# Autodesk Inventor assembly: tosaerba
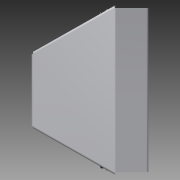
[picture p0: Inventor's stored thumbnail of the model, 180x180]
Saved by Autodesk Inventor 2014 SP2 (Build 180246200, 246)
## iProperties
Created: 2019-04-05
Part Number: tosaerba
Document SubType Name: Assembly
Designer: GauchoHP
Author: GauchoHP
## Documents named in this file (9)
- C:\Users\GauchoHP\Desktop\tosaerba\LawnmowerMechanicalProject\3D PROJECT - INVENTOR 2014\tosaerba.iam
- C:\Users\GauchoHP\Desktop\tosaerba\LawnmowerMechanicalProject\3D PROJECT - INVENTOR 2014\piastra.ipt
- C:\Users\GauchoHP\Desktop\tosaerba\LawnmowerMechanicalProject\3D PROJECT - INVENTOR 2014\motore.iam
- C:\Users\GauchoHP\Desktop\tosaerba\LawnmowerMechanicalProject\3D PROJECT - INVENTOR 2014\lama.ipt
- C:\Users\GauchoHP\Desktop\tosaerba\LawnmowerMechanicalProject\3D PROJECT - INVENTOR 2014\Imported Components\ruota pivottante\Assembly15.iam
- C:\Users\GauchoHP\Desktop\tosaerba\LawnmowerMechanicalProject\3D PROJECT - INVENTOR 2014\hoverboard naked.iam
- C:\Users\GauchoHP\Desktop\tosaerba\LawnmowerMechanicalProject\3D PROJECT - INVENTOR 2014\Imported Components\ruota pivottante\Assembly1.iam
- C:\Users\GauchoHP\Desktop\tosaerba\LawnmowerMechanicalProject\3D PROJECT - INVENTOR 2014\coverPolicarbonato2.ipt
- C:\Users\GauchoHP\Desktop\tosaerba\LawnmowerMechanicalProject\3D PROJECT - INVENTOR 2014\sponda laterale policarbonato.ipt
## Components (9 placed, 8 different names)
1. piastra:1 — Mate:8, Mate:37, Mate:43, Mate:45, Mate:46, Flush:3, Mate:47, Flush:4, Mate:48, Mate:49, Flush:5, Flush:6, Flush:7, Flush:8, Mate:50, Mate:51, Mate:52, Mate:53, Mate:54, Mate:55
2. motore:1 [sub-assembly] — Mate:8
3. lama:1 — Mate:43, Mate:53
4. Assembly15:1 [sub-assembly] — Mate:54, Mate:55
5. hoverboard naked:1 [sub-assembly] — Mate:37, Flush:2, Mate:48
6. Assembly1:1 [sub-assembly] — Mate:51, Mate:52
7. coverPolicarbonato2:1 — Flush:2, Mate:45, Mate:46, Flush:4
8. sponda laterale policarbonato:1 — Mate:49, Flush:5, Flush:6
9. sponda laterale policarbonato:2 — Flush:7, Flush:8, Mate:50
## Relationships (21: Mate 14, Flush 7)
- Mate:8: piastra:1 ↔ motore:1
- Mate:37: piastra:1 ↔ hoverboard naked:1
- Flush:2 (5.5 mm): hoverboard naked:1 ↔ coverPolicarbonato2:1
- Mate:43 (14 mm): piastra:1 ↔ lama:1
- Mate:45: piastra:1 ↔ coverPolicarbonato2:1
- Mate:46 (20 mm): piastra:1 ↔ coverPolicarbonato2:1
- Flush:3: piastra:1
- Mate:47 (66 mm): piastra:1
- Flush:4 (8 mm): piastra:1 ↔ coverPolicarbonato2:1
- Mate:48 (5 mm): piastra:1 ↔ hoverboard naked:1
- Mate:49: piastra:1 ↔ sponda laterale policarbonato:1
- Flush:5: piastra:1 ↔ sponda laterale policarbonato:1
- Flush:6 (20 mm): piastra:1 ↔ sponda laterale policarbonato:1
- Flush:7: piastra:1 ↔ sponda laterale policarbonato:2
- Flush:8 (-20 mm): piastra:1 ↔ sponda laterale policarbonato:2
- Mate:50: piastra:1 ↔ sponda laterale policarbonato:2
- Mate:51: piastra:1 ↔ Assembly1:1
- Mate:52: piastra:1 ↔ Assembly1:1
- Mate:53: piastra:1 ↔ lama:1
- Mate:54: piastra:1 ↔ Assembly15:1
- Mate:55: piastra:1 ↔ Assembly15:1
